# Autodesk Inventor assembly: canaletaMenor
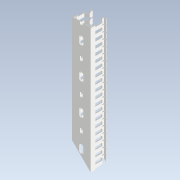
[picture p0: Inventor's stored thumbnail of the model, 180x180]
Saved by Autodesk Inventor 2021 (Build 250183000, 183)
## iProperties
Created: 2021-08-23
Part Number: canaletaMenor
Document SubType Name: Assembly
Designer: Andrés Holguín
Author: Andrés Holguín
## Documents named in this file (2)
- C:\Users\andre\Documents\GitHub\Dis.-Mecatronico-E6\inventor proyecto\Tablero\Canaletas\canaletaMenor.iam
- C:\Users\andre\Documents\GitHub\Dis.-Mecatronico-E6\inventor proyecto\Tablero\Canaletas\7308-1.iam
## Components (2 placed, 1 different names)
1. 7308-1:1 [sub-assembly] — Rigid:1, Mate:1, Angle:1, Mate:2, Angle:2
2. 7308-1:2 [sub-assembly] — Rigid:1
## Relationships (5: Mate 2, Angle 2, WeldJoint 1)
- Rigid:1 [WeldJoint]: 7308-1:1 ↔ 7308-1:2
- Mate:1: 7308-1:1
- Angle:1 (45 deg): 7308-1:1
- Mate:2: 7308-1:1
- Angle:2 (-45 deg): 7308-1:1
